# Autodesk Inventor assembly: 揺動節+ヘッケン
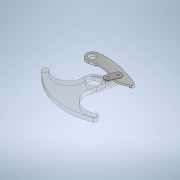
[picture p0: Inventor's stored thumbnail of the model, 180x180]
Saved by Autodesk Inventor 2022.2 (Build 262287000, 287)
## iProperties
Created: 2022-01-08
Part Number: 揺動節+ヘッケン
Document SubType Name: Assembly
Designer: acps
Author: acps
## Documents named in this file (4)
- C:\Users\acps\Documents\srdc\srdc_ksh\揺動節+ヘッケン.iam
- C:\Users\acps\Documents\srdc\srdc_ksh\揺動節.ipt
- C:\Users\acps\Documents\srdc\srdc_ksh\ヘッケン.ipt
- C:\Users\acps\Documents\srdc\srdc_ksh\ヘッケン抑え.ipt
## Components (3 placed, 3 different names)
1. 揺動節:1 — Mate:1, Insert:1, Mate:2
2. ヘッケン:1 — Mate:1, Insert:1, Insert:2, Mate:3
3. ヘッケン抑え:1 — Mate:2, Insert:2, Mate:3
## Relationships (5: Mate 3, Insert 2)
- Mate:1: 揺動節:1 ↔ ヘッケン:1
- Insert:1: 揺動節:1 ↔ ヘッケン:1
- Mate:2: 揺動節:1 ↔ ヘッケン抑え:1
- Insert:2: ヘッケン:1 ↔ ヘッケン抑え:1
- Mate:3: ヘッケン:1 ↔ ヘッケン抑え:1
